# Autodesk Inventor assembly: Ensamble herramienta
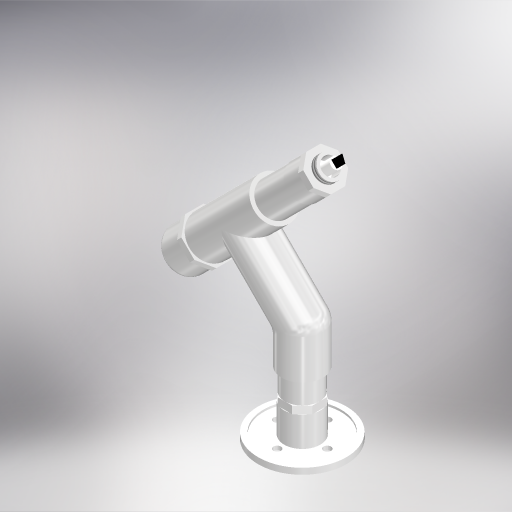
[picture p0: Inventor's stored thumbnail of the model, 512x512]
Saved by Autodesk Inventor 2023 (Build 270158000, 158)
## iProperties
Created: 2023-02-27
Part Number: Ensamble herramienta
Document SubType Name: Assembly
Designer: Braya
Mass: 162.999 g
Surface Area: 993.918 cm^2
Volume: 153.903 cm^3
Density: 1.0591 g/cm^3
Author: Braya
## Documents named in this file (12)
- C:\Users\Braya\OneDrive\Documentos\Universidad\Robótica\Laboratorio 1\Modelo\Ensamble herramienta.iam
- C:\Users\Braya\OneDrive\Documentos\Universidad\Robótica\Laboratorio 1\Modelo\Acople con rosca.ipt
- C:\Users\Braya\OneDrive\Documentos\Universidad\Robótica\Laboratorio 1\Modelo\Flanche.ipt
- C:\Users\Braya\OneDrive\Documentos\Universidad\Robótica\Laboratorio 1\Modelo\Semicodo.ipt
- C:\Users\Braya\OneDrive\Documentos\Universidad\Robótica\Laboratorio 1\Modelo\T.ipt
- C:\Users\Braya\OneDrive\Documentos\Universidad\Robótica\Laboratorio 1\Modelo\Tapón.ipt
- C:\Users\Braya\OneDrive\Documentos\Universidad\Robótica\Laboratorio 1\Modelo\Tubo 12 35.ipt
- C:\Users\Braya\OneDrive\Documentos\Universidad\Robótica\Laboratorio 1\Modelo\Tubo 34 20mm.ipt
- C:\Users\Braya\OneDrive\Documentos\Universidad\Robótica\Laboratorio 1\Modelo\Tubo 34 35mm.ipt
- C:\Users\Braya\OneDrive\Documentos\Universidad\Robótica\Laboratorio 1\Modelo\Tubo 12 40.ipt
- C:\Users\Braya\OneDrive\Documentos\Universidad\Robótica\Laboratorio 1\Modelo\Tubo 34 49mm.ipt
- C:\Users\Braya\OneDrive\Documentos\Universidad\Robótica\Laboratorio 1\Modelo\Marcador.ipt
## Components (13 placed, 11 different names)
1. Acople con rosca:1 — Coincidencia:2, Rígido:1, Rígido:2, Rígido:5
2. Flanche:1 — Nivelación:1, Nivelación:2, Nivelación:3, Coincidencia:2, Rígido:1
3. Semicodo:1 — Rígido:3, Rígido:5, Rígido:4, Coincidencia:3, Coincidencia:4
4. T:1 — Coincidencia:3, Coincidencia:4, Coincidencia:5, Rígido:6, Rígido:7, Rígido:10
5. Tapón:1 — Rígido:7
6. Tubo 12 35:1 — Rígido:2
7. Tubo 34 20mm:1 — Rígido:3
8. Tubo 34 35mm:1 — Rígido:4, Coincidencia:5
9. Tubo 34 35mm:2 — Rígido:6
10. Tubo 12 40:1 — Rígido:8
11. Tubo 34 49mm:1 — Rígido:9, Rígido:10
12. Acople con rosca:2 — Rígido:8, Rígido:9, De rotación:1, Coincidencia:6
13. Marcador:1 — De rotación:1, Coincidencia:6
## Relationships (19: WeldJoint 10, Mate 5, Flush 3, RevoluteJoint 1)
- Nivelación:1 [Flush]: Flanche:1
- Nivelación:2 [Flush]: Flanche:1
- Nivelación:3 [Flush]: Flanche:1
- Coincidencia:2 [Mate]: Acople con rosca:1 ↔ Flanche:1
- Rígido:1 [WeldJoint]: Acople con rosca:1 ↔ Flanche:1
- Rígido:2 [WeldJoint]: Acople con rosca:1 ↔ Tubo 12 35:1
- Rígido:3 [WeldJoint]: Semicodo:1 ↔ Tubo 34 20mm:1
- Rígido:5 [WeldJoint]: Acople con rosca:1 ↔ Semicodo:1
- Rígido:4 [WeldJoint]: Semicodo:1 ↔ Tubo 34 35mm:1
- Coincidencia:3 [Mate]: Semicodo:1 ↔ T:1
- Coincidencia:4 [Mate]: Semicodo:1 ↔ T:1
- Coincidencia:5 [Mate]: T:1 ↔ Tubo 34 35mm:1
- Rígido:6 [WeldJoint] (20 mm): T:1 ↔ Tubo 34 35mm:2
- Rígido:7 [WeldJoint]: T:1 ↔ Tapón:1
- Rígido:8 [WeldJoint]: Tubo 12 40:1 ↔ Acople con rosca:2
- Rígido:9 [WeldJoint]: Tubo 34 49mm:1 ↔ Acople con rosca:2
- Rígido:10 [WeldJoint] (15 mm): T:1 ↔ Tubo 34 49mm:1
- De rotación:1 [RevoluteJoint]: Acople con rosca:2 ↔ Marcador:1
- Coincidencia:6 [Mate]: Acople con rosca:2 ↔ Marcador:1
